# Autodesk Inventor assembly: head_assembly
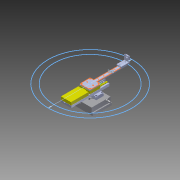
[picture p0: Inventor's stored thumbnail of the model, 180x180]
Saved by Autodesk Inventor 2011 (Build 150239000, 239)
## iProperties
Created: 2012-06-14
Part Number: head_assembly
Document SubType Name: Assembly
Designer: labuser
Author: labuser
## Documents named in this file (9)
- C:\Users\labuser\Desktop\cnc_cad\head_assembly.iam
- C:\Users\labuser\Desktop\cnc_cad\b_plate.ipt
- C:\Users\labuser\Desktop\cnc_cad\newport_SR50CC.ipt
- C:\Users\labuser\Desktop\cnc_cad\ripple_arm.ipt
- C:\Users\labuser\Desktop\cnc_cad\tdt_arm.ipt
- C:\Users\labuser\Desktop\cnc_cad\tdt_holder.ipt
- C:\Users\labuser\Desktop\cnc_cad\thorlabs_w_stage.ipt
- C:\Users\labuser\Desktop\cnc_cad\w_plate.ipt
- C:\Users\labuser\Desktop\cnc_cad\z_plate.ipt
## Components (8 placed, 8 different names)
1. b_plate:1 — Mate:8, Mate:9, Mate:11, Mate:12
2. newport_SR50CC:1 — Mate:11, Mate:12, Mate:13
3. ripple_arm:1 — Mate:1, Mate:4
4. tdt_arm:1 — Mate:1, Mate:2, Mate:3
5. tdt_holder:1 — Mate:2, Mate:3
6. thorlabs_w_stage:1 — Mate:4, Mate:7, Mate:10
7. w_plate:1 — Mate:7, Mate:8, Mate:9, Mate:10
8. z_plate:1 — Mate:13
## Relationships (11: Mate 11)
- Mate:1: ripple_arm:1 ↔ tdt_arm:1
- Mate:2: tdt_arm:1 ↔ tdt_holder:1
- Mate:3: tdt_arm:1 ↔ tdt_holder:1
- Mate:4: ripple_arm:1 ↔ thorlabs_w_stage:1
- Mate:7: thorlabs_w_stage:1 ↔ w_plate:1
- Mate:8: b_plate:1 ↔ w_plate:1
- Mate:9: b_plate:1 ↔ w_plate:1
- Mate:10: thorlabs_w_stage:1 ↔ w_plate:1
- Mate:11: b_plate:1 ↔ newport_SR50CC:1
- Mate:12: b_plate:1 ↔ newport_SR50CC:1
- Mate:13: newport_SR50CC:1 ↔ z_plate:1
